# Autodesk Inventor assembly: Assieme 1 - Trasporto
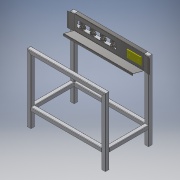
[picture p0: Inventor's stored thumbnail of the model, 180x180]
Saved by Autodesk Inventor 2018 (Build 220112000, 112)
## iProperties
Created: 2020-05-28
Part Number: Assieme 1 - Trasporto
Material: Generico
Document SubType Name: Assembly
Designer: Francesco
Author: Francesco
## Documents named in this file (6)
- C:\Users\Francesco\Desktop\Prova Inventor\Assieme 1 - Trasporto.iam
- C:\Users\Francesco\Desktop\Prova Inventor\Assieme tubolari.iam
- C:\Users\Francesco\Desktop\Prova Inventor\Lamiera riferimento.ipt
- C:\Users\Francesco\Desktop\Prova Inventor\Rullo con cuscinetti.iam
- C:\Users\Francesco\Desktop\Prova Inventor\Tubo.ipt
- C:\Users\Francesco\Desktop\Prova Inventor\Spessore plastica.ipt
## Components (8 placed, 5 different names)
1. Assieme tubolari:1 [sub-assembly] — Coincidente:1, Coincidente:2, Coincidente:3, Coincidente:4, Coincidente:5, Coincidente:6, Coincidente:7, Coincidente:8, Coincidente:9, Coincidente:10, Coincidente:11, Allineato:1
2. Lamiera riferimento:1 — Coincidente:1, Coincidente:2, Coincidente:3, Angolo:1, Coincidente:13, Coincidente:14, Coincidente:15
3. Rullo con cuscinetti:1 [sub-assembly] — Coincidente:8, Coincidente:11, Tangente:1
4. Rullo con cuscinetti:2 [sub-assembly] — Coincidente:4, Coincidente:5
5. Rullo con cuscinetti:3 [sub-assembly] — Coincidente:7, Coincidente:10
6. Rullo con cuscinetti:4 [sub-assembly] — Coincidente:6, Coincidente:9
7. Tubo:1 — Coincidente:12, Allineato:1
8. Spessore plastica:1 — Coincidente:13, Coincidente:14, Coincidente:15
## Relationships (18: Mate 15, Angle 1, Tangent 1, Flush 1)
- Coincidente:1 [Mate]: Assieme tubolari:1 ↔ Lamiera riferimento:1
- Coincidente:2 [Mate]: Assieme tubolari:1 ↔ Lamiera riferimento:1
- Coincidente:3 [Mate] (5 mm): Assieme tubolari:1 ↔ Lamiera riferimento:1
- Coincidente:4 [Mate]: Assieme tubolari:1 ↔ Rullo con cuscinetti:2
- Coincidente:5 [Mate]: Assieme tubolari:1 ↔ Rullo con cuscinetti:2
- Coincidente:6 [Mate]: Assieme tubolari:1 ↔ Rullo con cuscinetti:4
- Coincidente:7 [Mate]: Assieme tubolari:1 ↔ Rullo con cuscinetti:3
- Coincidente:8 [Mate]: Assieme tubolari:1 ↔ Rullo con cuscinetti:1
- Coincidente:9 [Mate]: Assieme tubolari:1 ↔ Rullo con cuscinetti:4
- Coincidente:10 [Mate]: Assieme tubolari:1 ↔ Rullo con cuscinetti:3
- Coincidente:11 [Mate]: Assieme tubolari:1 ↔ Rullo con cuscinetti:1
- Angolo:1 [Angle] (0 deg): Lamiera riferimento:1
- Tangente:1: Rullo con cuscinetti:1
- Coincidente:12 [Mate] (52 mm): Tubo:1
- Allineato:1 [Flush] (-1800 mm): Assieme tubolari:1 ↔ Tubo:1
- Coincidente:13 [Mate]: Lamiera riferimento:1 ↔ Spessore plastica:1
- Coincidente:14 [Mate]: Lamiera riferimento:1 ↔ Spessore plastica:1
- Coincidente:15 [Mate]: Lamiera riferimento:1 ↔ Spessore plastica:1
